# Autodesk Inventor assembly: Power brick assembly
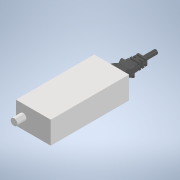
[picture p0: Inventor's stored thumbnail of the model, 180x180]
Saved by Autodesk Inventor 2022 (Build 260153000, 153)
## iProperties
Created: 2021-12-03
Part Number: Power brick assembly
Document SubType Name: Assembly
Designer: efred
Author: efred
## Documents named in this file (3)
- C:\Users\efred\OneDrive - Imperial College London\ROBOICP\Linear Rail Assembly\Power brick assembly.iam
- C:\Users\efred\OneDrive - Imperial College London\ROBOICP\Linear Rail Assembly\Power brick.ipt
- C:\Users\efred\OneDrive - Imperial College London\ROBOICP\Linear Rail Assembly\IEC 320 C13 Cable End.ipt
## Components (2 placed, 2 different names)
1. Power brick:1 — Mate:1, Flush:1, Flush:2
2. IEC 320 C13 Cable End:1 — Mate:1, Flush:1, Flush:2
## Relationships (3: Flush 2, Mate 1)
- Mate:1: Power brick:1 ↔ IEC 320 C13 Cable End:1
- Flush:1 (14 mm): Power brick:1 ↔ IEC 320 C13 Cable End:1
- Flush:2 (9 mm): Power brick:1 ↔ IEC 320 C13 Cable End:1
